# Autodesk Inventor assembly: PhotoBoothFrame
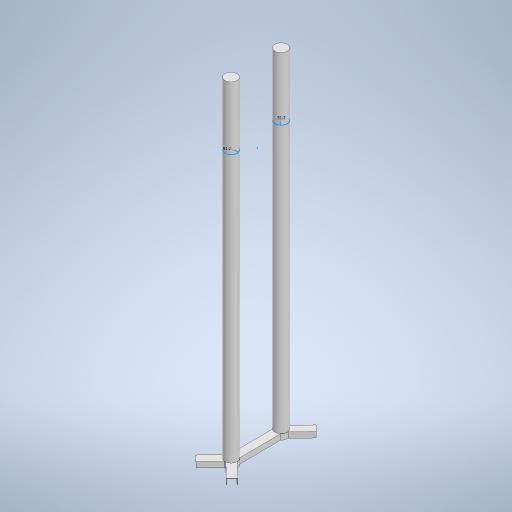
[picture p0: Inventor's stored thumbnail of the model, 512x512]
Saved by Autodesk Inventor 2023.1 (Build 271208000, 208)
## iProperties
Created: 2023-07-08
Part Number: PhotoBoothFrame
Document SubType Name: Assembly
Designer: Robot
Author: Robot
## Documents named in this file (4)
- C:\Users\Robot\Documents\PhotoBoothFrame\PhotoBoothFrame.iam
- C:\Users\Robot\Documents\PhotoBoothFrame\Tube.ipt
- C:\Users\Robot\Documents\PhotoBoothFrame\Base.ipt
- C:\Users\Robot\Documents\CameraBracket.ipt
## Components (4 placed, 3 different names)
1. Tube:1 — Flush:1, Mate:1, Mate:2
2. Tube:2 — Mate:3, Mate:4, Flush:2
3. Base:1 — Flush:1, Mate:1, Mate:2, Mate:3, Mate:4
4. CameraBracket:1 — Flush:2
## Relationships (6: Mate 4, Flush 2)
- Flush:1: Tube:1 ↔ Base:1
- Mate:1: Tube:1 ↔ Base:1
- Mate:2: Tube:1 ↔ Base:1
- Mate:3: Tube:2 ↔ Base:1
- Mate:4: Tube:2 ↔ Base:1
- Flush:2 (-262.25 mm): Tube:2 ↔ CameraBracket:1
